# Autodesk Inventor assembly: Сборка
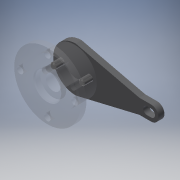
[picture p0: Inventor's stored thumbnail of the model, 180x180]
Saved by Autodesk Inventor 2019.3 (Build 233278000, 278)
## iProperties
Created: 2020-04-04
Part Number: Сборка
Material: Типовые
Document SubType Name: Assembly
Designer: Admin
Mass: 349.084 g
Surface Area: 611.86 cm^2
Volume: 313.659 cm^3
Density: 1.11294 g/cm^3
Author: Admin
## Documents named in this file (4)
- D:\МГТУ Учеба\2 Семестр\Инжграф\Модуль 3\Диана\Сборка.iam
- D:\МГТУ Учеба\2 Семестр\Инжграф\Модуль 3\Диана\Фланец.ipt
- D:\МГТУ Учеба\2 Семестр\Инжграф\Модуль 3\Диана\Рычаг.ipt
- C:\Users\Admin\Documents\Inventor\Content Center Files\R2019\ru-RU\GOST 17474-80 (1)\Винт M10-6gx25 ГОСТ 17474-80.ipt
## Components (4 placed, 3 different names)
1. Фланец:1 — Совмещение:1, Совмещение:2, Совмещение:3
2. Рычаг:1 — Совмещение:1, Совмещение:2, Совмещение:3, Совмещение:5, Совмещение:6
3. Винт ГОСТ 17474-80 M10 x 25:2 — Совмещение:5
4. Винт ГОСТ 17474-80 M10 x 25:3 — Совмещение:6
## Relationships (5: Mate 5)
- Совмещение:1 [Mate]: Фланец:1 ↔ Рычаг:1
- Совмещение:2 [Mate]: Фланец:1 ↔ Рычаг:1
- Совмещение:3 [Mate]: Фланец:1 ↔ Рычаг:1
- Совмещение:5 [Mate]: Рычаг:1 ↔ Винт ГОСТ 17474-80 M10 x 25:2
- Совмещение:6 [Mate]: Рычаг:1 ↔ Винт ГОСТ 17474-80 M10 x 25:3
